# Autodesk Inventor assembly: Assembly
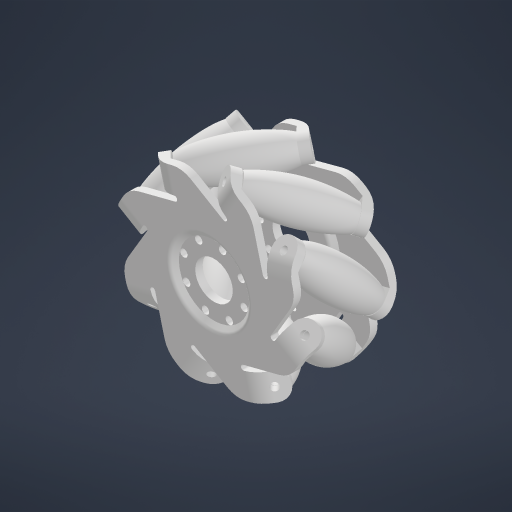
[picture p0: Inventor's stored thumbnail of the model, 512x512]
Saved by Autodesk Inventor 2023 (Build 270158000, 158)
## iProperties
Created: 2023-04-05
Part Number: Assembly
Document SubType Name: Assembly
Designer: vatdu
Author: vatdu
## Documents named in this file (3)
- C:\Users\vatdu\Desktop\CRYSTAL MARK I\Wheels\Assembly.iam
- C:\Users\vatdu\Desktop\CRYSTAL MARK I\Wheels\Roller V3.ipt
- C:\Users\vatdu\Desktop\CRYSTAL MARK I\Wheels\Frame V2.ipt
## Components (10 placed, 2 different names)
1. Roller V3:1 — Rotational:4
2. Roller V3:2 — Rotational:5
3. Roller V3:3 — Rotational:6
4. Roller V3:4 — Rotational:7
5. Roller V3:5 — Rotational:8
6. Roller V3:6 — Rotational:3
7. Roller V3:7 — Rotational:2
8. Roller V3:8 — Rotational:1
9. Frame V2:1 — Rotational:1, Rotational:2, Rotational:3, Rotational:4, Rotational:5, Rotational:6, Rotational:7, Rotational:8
10. Frame V2:2
## Relationships (8: RevoluteJoint 8)
- Rotational:1 [RevoluteJoint]: Roller V3:8 ↔ Frame V2:1
- Rotational:2 [RevoluteJoint]: Roller V3:7 ↔ Frame V2:1
- Rotational:3 [RevoluteJoint]: Roller V3:6 ↔ Frame V2:1
- Rotational:4 [RevoluteJoint]: Roller V3:1 ↔ Frame V2:1
- Rotational:5 [RevoluteJoint]: Roller V3:2 ↔ Frame V2:1
- Rotational:6 [RevoluteJoint]: Roller V3:3 ↔ Frame V2:1
- Rotational:7 [RevoluteJoint]: Roller V3:4 ↔ Frame V2:1
- Rotational:8 [RevoluteJoint]: Roller V3:5 ↔ Frame V2:1
